# Autodesk Inventor assembly: generaqtor-assembly
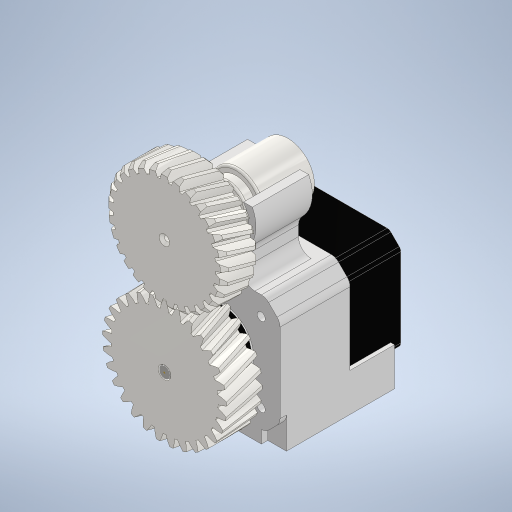
[picture p0: Inventor's stored thumbnail of the model, 512x512]
Saved by Autodesk Inventor 2024.1 (Build 281209000, 209)
## iProperties
Created: 2026-03-30
Part Number: generaqtor-assembly
Document SubType Name: Assembly
Designer: iwheard
Author: iwheard
## Documents named in this file (3)
- C:\Users\iwheard\Documents\0004-CAD\3D-cad-main\u-stepper-generator\generaqtor-assembly.iam
- C:\Users\iwheard\Documents\0004-CAD\3D-cad-main\u-stepper-generator\ustepper-generator.ipt
- C:\Users\iwheard\Documents\0004-CAD\3D-cad-main\u-stepper-generator\generaqtor-assembly\Design Accelerator\Spur Gears3.iam
## Components (2 placed, 2 different names)
1. ustepper-generator:1 — Mate:1, Flush:1
2. Spur Gears:1 [sub-assembly] — Mate:1, Flush:1
## Relationships (2: Mate 1, Flush 1)
- Mate:1: ustepper-generator:1 ↔ Spur Gears:1
- Flush:1: ustepper-generator:1 ↔ Spur Gears:1
